# Autodesk Inventor assembly: Gears
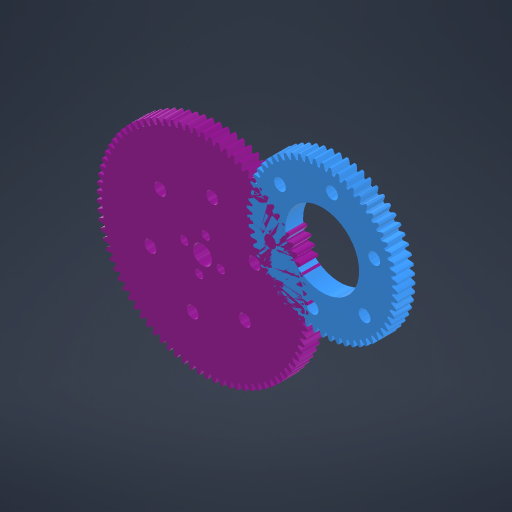
[picture p0: Inventor's stored thumbnail of the model, 512x512]
Saved by Autodesk Inventor 2024.2 (Build 282272000, 272)
## iProperties
Created: 2023-01-07
Part Number: Gears
Document SubType Name: Assembly
Designer: Allan
Author: Allan
## Documents named in this file (4)
- C:\Users\alniles07\Documents\Github\8400_2024_CAD\Gears.iam
- C:\Users\alniles07\Documents\Github\8400_2024_CAD\FTC Wheel Motor Gear.ipt
- C:\Users\alniles07\Documents\Github\8400_2024_CAD\FTC Wheel Gear.ipt
- C:\Users\Jason\Documents\Inventor\FTC Robot 2023\Gears\Design Accelerator\Spur Gears1.iam
## Components (3 placed, 3 different names)
1. Spur Gear1:1 — Mate:1, Mate:2
2. Spur Gear2:1 — Mate:3, Mate:4
3. Spur Gears:1 [sub-assembly] — Mate:1, Mate:2, Mate:3, Mate:4
## Relationships (4: Mate 4)
- Mate:1: Spur Gear1:1 ↔ Spur Gears:1
- Mate:2: Spur Gear1:1 ↔ Spur Gears:1
- Mate:3: Spur Gear2:1 ↔ Spur Gears:1
- Mate:4: Spur Gear2:1 ↔ Spur Gears:1
